# Autodesk Inventor assembly: Assembly Rack_2
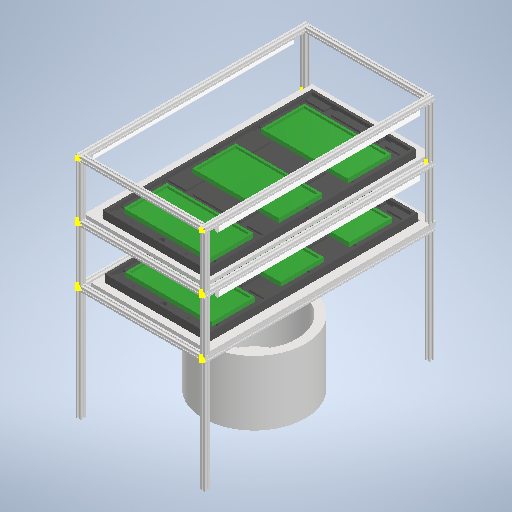
[picture p0: Inventor's stored thumbnail of the model, 512x512]
Saved by Autodesk Inventor 2025 (Build 290162000, 162)
## iProperties
Created: 2024-07-12
Part Number: Assembly Rack_2
Document SubType Name: Assembly
Designer: User
Author: User
## Documents named in this file (10)
- C:\Users\User\OneDrive\Documents\FYP\Inventor_Designs\Rack\Assembly Rack_2.iam
- C:\Users\User\OneDrive\Documents\FYP\Inventor_Designs\Rack\Metal_Profile 70cm.ipt
- C:\Users\User\OneDrive\Documents\FYP\Inventor_Designs\Rack\Metal_Profile 135cm.ipt
- C:\Users\User\OneDrive\Documents\FYP\Inventor_Designs\Rack\Metal Profile 30 cm.ipt
- C:\Users\User\OneDrive\Documents\FYP\Inventor_Designs\Rack\Metal_Profile 65 cm.ipt
- C:\Users\User\OneDrive\Documents\FYP\Inventor_Designs\Rack\Light tube 118.4cm.ipt
- C:\Users\User\OneDrive\Documents\FYP\Inventor_Designs\Rack\Part3.ipt
- C:\Users\User\OneDrive\Documents\FYP\Inventor_Designs\Rack\flood tray.ipt
- C:\Users\User\OneDrive\Documents\FYP\Inventor_Designs\Rack\Tub.ipt
- C:\Users\User\OneDrive\Documents\FYP\Inventor_Designs\Platform\Potting Tray.ipt
## Components (39 placed, 9 different names)
1. Metal_Profile 70cm:1 — Mate:1, Flush:1, Flush:2, Mate:2, Flush:3, Flush:4, Flush:63, Flush:67
2. Metal_Profile 70cm:2 — Mate:3, Flush:5, Flush:6, Flush:7, Flush:8
3. Metal_Profile 135cm:1 — Mate:1, Flush:1, Flush:2, Mate:3, Flush:5, Flush:6, Mate:11, Flush:25, Flush:26, Mate:20, Flush:49, Flush:50, Mate:22, Flush:53, Flush:54, Flush:64, Mate:33, Flush:68
4. Metal_Profile 135cm:2 — Mate:2, Flush:3, Flush:4, Flush:7, Flush:8, Flush:27, Flush:28, Mate:21, Flush:51, Flush:52, Mate:23, Flush:55, Flush:56
5. Metal_Profile 70cm:3 — Flush:61, Flush:65
6. Metal_Profile 70cm:4
7. Metal_Profile 135cm:3 — Mate:7, Flush:17, Flush:18, Mate:9, Flush:21, Flush:22, Mate:19, Flush:45, Flush:46, Mate:26, Flush:58, Flush:62, Mate:32, Flush:66
8. Metal_Profile 135cm:4 — Mate:8, Flush:19, Flush:20, Mate:10, Flush:23, Flush:24, Flush:47, Flush:48, Mate:30, Flush:60
9. Metal Profile 30 cm:1 — Mate:7, Flush:17, Flush:18, Mate:11, Flush:25, Flush:26, Mate:27
10. Metal Profile 30 cm:2 — Mate:9, Flush:21, Flush:22
11. Metal Profile 30 cm:3 — Mate:10, Flush:23, Flush:24
12. Metal Profile 30 cm:4 — Mate:8, Flush:19, Flush:20, Flush:27, Flush:28, Mate:31
13. Metal_Profile 70cm:5
14. Metal_Profile 70cm:6
15. Metal_Profile 135cm:5 — Mate:24, Flush:57
16. Metal_Profile 135cm:6 — Mate:28, Flush:59
17. Metal Profile 30 cm:5 — Mate:19, Flush:45, Flush:46, Mate:25
18. Metal Profile 30 cm:6
19. Metal Profile 30 cm:7
20. Metal Profile 30 cm:8 — Flush:47, Flush:48, Mate:29
21. Metal_Profile 65 cm:1 — Mate:21, Flush:51, Flush:52
22. Metal_Profile 65 cm:2 — Mate:23, Flush:55, Flush:56
23. Metal_Profile 65 cm:3 — Mate:20, Flush:49, Flush:50, Flush:69
24. Metal_Profile 65 cm:4 — Mate:22, Flush:53, Flush:54
25. Light tube 118.4cm:1 — Mate:28, Flush:59, Mate:29
26. Light tube 118.4cm:2 — Mate:26, Flush:58, Mate:27
27. Light tube 118.4cm:3 — Mate:24, Flush:57, Mate:25
28. Light tube 118.4cm:4 — Mate:30, Flush:60, Mate:31
29. Part3:1 — Flush:63, Flush:64, Mate:33, Mate:35
30. Part3:2 — Flush:61, Flush:62, Mate:32, Mate:34
31. flood tray:6 — Mate:34, Flush:65, Flush:66, Mate:36, Mate:37, Mate:38, Mate:42, Mate:43, Mate:44, Mate:46
32. flood tray:7 — Mate:35, Flush:67, Flush:68, Mate:39, Mate:40, Mate:41, Mate:48, Mate:49, Mate:50, Mate:52
33. Tub:1 — Flush:69
34. Potting Tray:1 — Mate:37, Mate:44, Mate:45, Mate:47
35. Potting Tray:2 — Mate:38, Mate:46, Mate:47
36. Potting Tray:3 — Mate:36, Mate:42, Mate:43, Mate:45
37. Potting Tray:4 — Mate:39, Mate:48, Mate:49, Mate:51
38. Potting Tray:5 — Mate:40, Mate:50, Mate:51, Mate:53
39. Potting Tray:6 — Mate:41, Mate:52, Mate:53
## Relationships (122: Flush 69, Mate 53)
- Mate:1: Metal_Profile 70cm:1 ↔ Metal_Profile 135cm:1
- Flush:1: Metal_Profile 70cm:1 ↔ Metal_Profile 135cm:1
- Flush:2: Metal_Profile 70cm:1 ↔ Metal_Profile 135cm:1
- Mate:2: Metal_Profile 70cm:1 ↔ Metal_Profile 135cm:2
- Flush:3: Metal_Profile 70cm:1 ↔ Metal_Profile 135cm:2
- Flush:4: Metal_Profile 70cm:1 ↔ Metal_Profile 135cm:2
- Mate:3: Metal_Profile 70cm:2 ↔ Metal_Profile 135cm:1
- Flush:5: Metal_Profile 70cm:2 ↔ Metal_Profile 135cm:1
- Flush:6: Metal_Profile 70cm:2 ↔ Metal_Profile 135cm:1
- Flush:7: Metal_Profile 70cm:2 ↔ Metal_Profile 135cm:2
- Flush:8: Metal_Profile 70cm:2 ↔ Metal_Profile 135cm:2
- [Mate]: Metal_Profile 70cm:3 ↔ Metal_Profile 135cm:3
- [Flush]: Metal_Profile 70cm:3 ↔ Metal_Profile 135cm:3
- [Flush]: Metal_Profile 70cm:3 ↔ Metal_Profile 135cm:3
- [Mate]: Metal_Profile 70cm:3 ↔ Metal_Profile 135cm:4
- [Flush]: Metal_Profile 70cm:3 ↔ Metal_Profile 135cm:4
- [Flush]: Metal_Profile 70cm:3 ↔ Metal_Profile 135cm:4
- [Mate]: Metal_Profile 70cm:4 ↔ Metal_Profile 135cm:3
- [Flush]: Metal_Profile 70cm:4 ↔ Metal_Profile 135cm:3
- [Flush]: Metal_Profile 70cm:4 ↔ Metal_Profile 135cm:3
- [Flush]: Metal_Profile 70cm:4 ↔ Metal_Profile 135cm:4
- [Flush]: Metal_Profile 70cm:4 ↔ Metal_Profile 135cm:4
- Mate:7: Metal_Profile 135cm:3 ↔ Metal Profile 30 cm:1
- Flush:17: Metal_Profile 135cm:3 ↔ Metal Profile 30 cm:1
- Flush:18: Metal_Profile 135cm:3 ↔ Metal Profile 30 cm:1
- Mate:8: Metal_Profile 135cm:4 ↔ Metal Profile 30 cm:4
- Flush:19: Metal_Profile 135cm:4 ↔ Metal Profile 30 cm:4
- Flush:20: Metal_Profile 135cm:4 ↔ Metal Profile 30 cm:4
- Mate:9: Metal_Profile 135cm:3 ↔ Metal Profile 30 cm:2
- Flush:21: Metal_Profile 135cm:3 ↔ Metal Profile 30 cm:2
- Flush:22: Metal_Profile 135cm:3 ↔ Metal Profile 30 cm:2
- Mate:10: Metal_Profile 135cm:4 ↔ Metal Profile 30 cm:3
- Flush:23: Metal_Profile 135cm:4 ↔ Metal Profile 30 cm:3
- Flush:24: Metal_Profile 135cm:4 ↔ Metal Profile 30 cm:3
- Mate:11: Metal_Profile 135cm:1 ↔ Metal Profile 30 cm:1
- Flush:25: Metal_Profile 135cm:1 ↔ Metal Profile 30 cm:1
- Flush:26: Metal_Profile 135cm:1 ↔ Metal Profile 30 cm:1
- Flush:27: Metal_Profile 135cm:2 ↔ Metal Profile 30 cm:4
- Flush:28: Metal_Profile 135cm:2 ↔ Metal Profile 30 cm:4
- [Mate]: Metal_Profile 70cm:5 ↔ Metal_Profile 135cm:5
- [Flush]: Metal_Profile 70cm:5 ↔ Metal_Profile 135cm:5
- [Flush]: Metal_Profile 70cm:5 ↔ Metal_Profile 135cm:5
- [Mate]: Metal_Profile 70cm:5 ↔ Metal_Profile 135cm:6
- [Flush]: Metal_Profile 70cm:5 ↔ Metal_Profile 135cm:6
- [Flush]: Metal_Profile 70cm:5 ↔ Metal_Profile 135cm:6
- [Mate]: Metal_Profile 70cm:6 ↔ Metal_Profile 135cm:5
- [Flush]: Metal_Profile 70cm:6 ↔ Metal_Profile 135cm:5
- [Flush]: Metal_Profile 70cm:6 ↔ Metal_Profile 135cm:5
- [Flush]: Metal_Profile 70cm:6 ↔ Metal_Profile 135cm:6
- [Flush]: Metal_Profile 70cm:6 ↔ Metal_Profile 135cm:6
- [Mate]: Metal_Profile 135cm:5 ↔ Metal Profile 30 cm:5
- [Flush]: Metal_Profile 135cm:5 ↔ Metal Profile 30 cm:5
- [Flush]: Metal_Profile 135cm:5 ↔ Metal Profile 30 cm:5
- [Mate]: Metal_Profile 135cm:6 ↔ Metal Profile 30 cm:8
- [Flush]: Metal_Profile 135cm:6 ↔ Metal Profile 30 cm:8
- [Flush]: Metal_Profile 135cm:6 ↔ Metal Profile 30 cm:8
- [Mate]: Metal_Profile 135cm:5 ↔ Metal Profile 30 cm:6
- [Flush]: Metal_Profile 135cm:5 ↔ Metal Profile 30 cm:6
- [Flush]: Metal_Profile 135cm:5 ↔ Metal Profile 30 cm:6
- [Mate]: Metal_Profile 135cm:6 ↔ Metal Profile 30 cm:7
- [Flush]: Metal_Profile 135cm:6 ↔ Metal Profile 30 cm:7
- [Flush]: Metal_Profile 135cm:6 ↔ Metal Profile 30 cm:7
- Mate:19: Metal_Profile 135cm:3 ↔ Metal Profile 30 cm:5
- Flush:45: Metal_Profile 135cm:3 ↔ Metal Profile 30 cm:5
- Flush:46: Metal_Profile 135cm:3 ↔ Metal Profile 30 cm:5
- Flush:47: Metal_Profile 135cm:4 ↔ Metal Profile 30 cm:8
- Flush:48: Metal_Profile 135cm:4 ↔ Metal Profile 30 cm:8
- Mate:20: Metal_Profile 135cm:1 ↔ Metal_Profile 65 cm:3
- Flush:49: Metal_Profile 135cm:1 ↔ Metal_Profile 65 cm:3
- Flush:50: Metal_Profile 135cm:1 ↔ Metal_Profile 65 cm:3
- Mate:21: Metal_Profile 135cm:2 ↔ Metal_Profile 65 cm:1
- Flush:51: Metal_Profile 135cm:2 ↔ Metal_Profile 65 cm:1
- Flush:52: Metal_Profile 135cm:2 ↔ Metal_Profile 65 cm:1
- Mate:22: Metal_Profile 135cm:1 ↔ Metal_Profile 65 cm:4
- Flush:53: Metal_Profile 135cm:1 ↔ Metal_Profile 65 cm:4
- Flush:54: Metal_Profile 135cm:1 ↔ Metal_Profile 65 cm:4
- Mate:23: Metal_Profile 135cm:2 ↔ Metal_Profile 65 cm:2
- Flush:55: Metal_Profile 135cm:2 ↔ Metal_Profile 65 cm:2
- Flush:56: Metal_Profile 135cm:2 ↔ Metal_Profile 65 cm:2
- Mate:24: Metal_Profile 135cm:5 ↔ Light tube 118.4cm:3
- Flush:57: Metal_Profile 135cm:5 ↔ Light tube 118.4cm:3
- Mate:25 (50 mm): Metal Profile 30 cm:5 ↔ Light tube 118.4cm:3
- Mate:26: Metal_Profile 135cm:3 ↔ Light tube 118.4cm:2
- Flush:58: Metal_Profile 135cm:3 ↔ Light tube 118.4cm:2
- Mate:27 (50 mm): Metal Profile 30 cm:1 ↔ Light tube 118.4cm:2
- Mate:28: Metal_Profile 135cm:6 ↔ Light tube 118.4cm:1
- Flush:59: Metal_Profile 135cm:6 ↔ Light tube 118.4cm:1
- Mate:29 (50 mm): Metal Profile 30 cm:8 ↔ Light tube 118.4cm:1
- Mate:30: Metal_Profile 135cm:4 ↔ Light tube 118.4cm:4
- Flush:60: Metal_Profile 135cm:4 ↔ Light tube 118.4cm:4
- Mate:31 (50 mm): Metal Profile 30 cm:4 ↔ Light tube 118.4cm:4
- Flush:61 (30 mm): Metal_Profile 70cm:3 ↔ Part3:2
- Flush:62 (30 mm): Metal_Profile 135cm:3 ↔ Part3:2
- Mate:32: Metal_Profile 135cm:3 ↔ Part3:2
- Flush:63 (30 mm): Metal_Profile 70cm:1 ↔ Part3:1
- Flush:64: Metal_Profile 135cm:1 ↔ Part3:1
- Mate:33: Metal_Profile 135cm:1 ↔ Part3:1
- Mate:34: Part3:2 ↔ flood tray:6
- Flush:65 (60 mm): Metal_Profile 70cm:3 ↔ flood tray:6
- Flush:66 (50 mm): Metal_Profile 135cm:3 ↔ flood tray:6
- Mate:35: Part3:1 ↔ flood tray:7
- Flush:67 (70 mm): Metal_Profile 70cm:1 ↔ flood tray:7
- Flush:68 (50 mm): Metal_Profile 135cm:1 ↔ flood tray:7
- Flush:69: Metal_Profile 65 cm:3 ↔ Tub:1
- Mate:36: flood tray:6 ↔ Potting Tray:3
- Mate:37: flood tray:6 ↔ Potting Tray:1
- Mate:38: flood tray:6 ↔ Potting Tray:2
- Mate:39: flood tray:7 ↔ Potting Tray:4
- Mate:40: flood tray:7 ↔ Potting Tray:5
- Mate:41: flood tray:7 ↔ Potting Tray:6
- Mate:42 (30 mm): flood tray:6 ↔ Potting Tray:3
- Mate:43 (50 mm): flood tray:6 ↔ Potting Tray:3
- Mate:44 (30 mm): flood tray:6 ↔ Potting Tray:1
- Mate:45 (150 mm): Potting Tray:1 ↔ Potting Tray:3
- Mate:46 (30 mm): flood tray:6 ↔ Potting Tray:2
- Mate:47 (150 mm): Potting Tray:1 ↔ Potting Tray:2
- Mate:48 (30 mm): flood tray:7 ↔ Potting Tray:4
- Mate:49 (50 mm): flood tray:7 ↔ Potting Tray:4
- Mate:50 (30 mm): flood tray:7 ↔ Potting Tray:5
- Mate:51 (150 mm): Potting Tray:4 ↔ Potting Tray:5
- Mate:52 (30 mm): flood tray:7 ↔ Potting Tray:6
- Mate:53 (150 mm): Potting Tray:5 ↔ Potting Tray:6
## Named parameters: d11_d0 = 0 mm, d12_d1 = 0 mm, d13_d2 = 0 mm, d14_d3 = 0 mm, d15_d4 = 0 mm, d16_d5 = 0 mm, d17_d6 = 0 mm, d18_d7 = 0 mm, d19_d8 = 0 mm, d20_d9 = 0 mm, d21_d10 = 0 mm, d39_d22 = 0 mm, d40_d23 = 0 mm, d41_d24 = 0 mm, d42_d25 = 0 mm, d43_d26 = 0 mm, d44_d27 = 0 mm, d45_d28 = 0 mm, d46_d29 = 0 mm, d47_d30 = 0 mm, d48_d31 = 0 mm, d49_d11_d0 = 0 mm, d50_d12_d1 = 0 mm, d51_d13_d2 = 0 mm, d52_d14_d3 = 0 mm, d53_d15_d4 = 0 mm, d54_d16_d5 = 0 mm, d55_d17_d6 = 0 mm, d56_d18_d7 = 0 mm, d57_d19_d8 = 0 mm, d58_d20_d9 = 0 mm, d59_d21_d10 = 0 mm, d60_d32 = 0 mm, d61_d33 = 0 mm
